# Autodesk Inventor assembly: Assembly
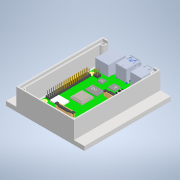
[picture p0: Inventor's stored thumbnail of the model, 180x180]
Saved by Autodesk Inventor 2020 (Build 240168000, 168)
## iProperties
Created: 2020-01-18
Part Number: Assembly
Document SubType Name: Assembly
Designer: chris
Author: chris
## Documents named in this file (3)
- D:\Projects\Casserole\RobotCasserole2020\piVisionCase\Assembly.iam
- D:\Projects\Casserole\RobotCasserole2020\piVisionCase\Raspberry Pi 4 Model B.iam
- D:\Projects\Casserole\RobotCasserole2020\piVisionCase\bottom.ipt
## Components (2 placed, 2 different names)
1. Raspberry Pi 4 Model B:1 [sub-assembly] — Insert:1, Angle:1
2. bottom:1 — Insert:1, Angle:1
## Relationships (2: Insert 1, Angle 1)
- Insert:1: Raspberry Pi 4 Model B:1 ↔ bottom:1
- Angle:1 (180 deg): Raspberry Pi 4 Model B:1 ↔ bottom:1
